# Autodesk Inventor assembly: Baugruppe1
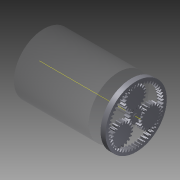
[picture p0: Inventor's stored thumbnail of the model, 180x180]
Saved by Autodesk Inventor 2014 (Build 180170000, 170)
## iProperties
Created: 2013-05-23
Part Number: Baugruppe1
Document SubType Name: Assembly
Designer: hartmann
Author: hartmann
## Documents named in this file (6)
- C:\Dokumente und Einstellungen\hartmann\Desktop\Beep\Hardware\Model2\Getriebe1.iam
- Getriebe1.iam
- C:\Dokumente und Einstellungen\hartmann\Desktop\Beep\Hardware\Model2\motor.ipt
- C:\Dokumente und Einstellungen\hartmann\Desktop\Beep\Hardware\Model2\Getriebe1\Konstruktions-Assistent\Stirnräder1.iam
- C:\Dokumente und Einstellungen\hartmann\Desktop\Beep\Hardware\Model2\Getriebe1\Konstruktions-Assistent\Stirnräder2.iam
- C:\Dokumente und Einstellungen\hartmann\Desktop\Beep\Hardware\Model2\Getriebe1\Konstruktions-Assistent\Stirnräder3.iam
## Components (6 placed, 2 different names)
1. motor:1 — Passend:1
2. Stirnräder:1 [sub-assembly]
3. Stirnräder:3 [sub-assembly] — Passend:4
4. Stirnräder:2 [sub-assembly]
5. Stirnräder:4 [sub-assembly]
6. Stirnräder:5 [sub-assembly]
## Component patterns: (3 elements, first: Stirnräder:2)
## Relationships (2: Mate 2)
- Passend:1 [Mate]: motor:1
- Passend:4 [Mate]: Stirnräder:3
